# Autodesk Inventor assembly: A1
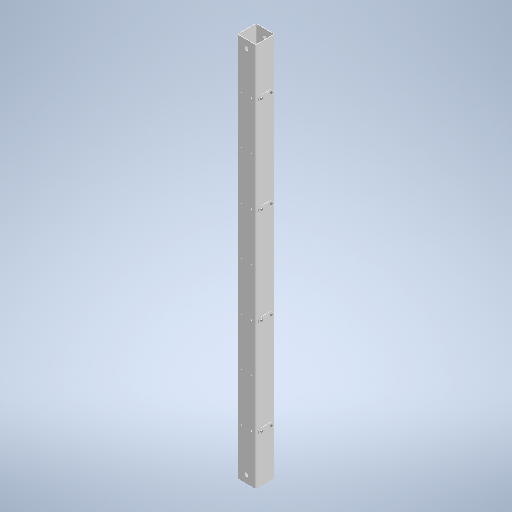
[picture p0: Inventor's stored thumbnail of the model, 512x512]
Saved by Autodesk Inventor 2025.2 (Build 292293000, 293)
## iProperties
Created: 2025-03-24
Part Number: A1
Document SubType Name: Assembly
Designer: Caspe
Author: Caspe
## Documents named in this file (6)
- C:\Users\Caspe\Documents\Semester 8\Project\Anomaly_Detection\Mechanical_Project\Inventor_project\A1.iam
- C:\Users\Caspe\Documents\Semester 8\Project\Anomaly_Detection\Mechanical_Project\Inventor_project\A1_Beam.ipt
- C:\Users\Caspe\Documents\Semester 8\Project\Anomaly_Detection\Mechanical_Project\Inventor_project\A1_joiners.ipt
- C:\Users\Caspe\Documents\Inventor\Content Center Files\R2025\en-US\Blind Rivet GB_T 12615.1-2004\Blind Rivet GB_T 12615.1-2004 3.2 X 10.5.ipt
- C:\Users\Caspe\Documents\Semester 8\Project\Anomaly_Detection\Mechanical_Project\Inventor_project\A1_joiners_MIR.ipt
- C:\Users\Caspe\Documents\Semester 8\Project\Anomaly_Detection\Mechanical_Project\Inventor_project\Leg_press_parameters.xlsx
## Components (26 placed, 4 different names)
1. A1_Beam:1 — Mate:1, Mate:2, Mate:3, Mate:4, Mate:6
2. A1_Beam:2 — Mate:1, Mate:2, Mate:3, Mate:5
3. A1_joiners_MIR:1 — Insert:2
4. A1_joiners_MIR:2
5. Blind Rivet GB/T 12615.1-2004 3.2 X 10.5:10
6. Blind Rivet GB/T 12615.1-2004 3.2 X 10.5:11
7. A1_joiners_MIR:3
8. Blind Rivet GB/T 12615.1-2004 3.2 X 10.5:12
9. Blind Rivet GB/T 12615.1-2004 3.2 X 10.5:13
10. A1_joiners_MIR:4
11. Blind Rivet GB/T 12615.1-2004 3.2 X 10.5:14
12. Blind Rivet GB/T 12615.1-2004 3.2 X 10.5:15
13. A1_joiners:1 — Mate:4, Mate:5, Mate:6, Insert:1
14. A1_joiners:2
15. A1_joiners:3
16. A1_joiners:4
17. Blind Rivet GB/T 12615.1-2004 3.2 X 10.5:9 — Insert:2
18. Blind Rivet GB/T 12615.1-2004 3.2 X 10.5:16
19. Blind Rivet GB/T 12615.1-2004 3.2 X 10.5:1 — Insert:1
20. Blind Rivet GB/T 12615.1-2004 3.2 X 10.5:2
21. Blind Rivet GB/T 12615.1-2004 3.2 X 10.5:3
22. Blind Rivet GB/T 12615.1-2004 3.2 X 10.5:4
23. Blind Rivet GB/T 12615.1-2004 3.2 X 10.5:5
24. Blind Rivet GB/T 12615.1-2004 3.2 X 10.5:6
25. Blind Rivet GB/T 12615.1-2004 3.2 X 10.5:7
26. Blind Rivet GB/T 12615.1-2004 3.2 X 10.5:8
## Component patterns: (4 elements, first: A1_joiners:1), (2 elements, first: Blind Rivet GB/T 12615.1-2004 3.2 X 10.5:9), (2 elements, first: Blind Rivet GB/T 12615.1-2004 3.2 X 10.5:1), Component Pattern 1:2 (2 elements), Component Pattern 1:3 (2 elements), Component Pattern 1:4 (2 elements)
## Relationships (9: Mate 6, Insert 2, Flush 1)
- Mate:1: A1_Beam:1 ↔ A1_Beam:2
- Mate:2: A1_Beam:1 ↔ A1_Beam:2
- Mate:3: A1_Beam:1 ↔ A1_Beam:2
- Mate:4: A1_Beam:1 ↔ A1_joiners:1
- Mate:5: A1_Beam:2 ↔ A1_joiners:1
- Mate:6: A1_Beam:1 ↔ A1_joiners:1
- Insert:1: A1_joiners:1 ↔ Blind Rivet GB/T 12615.1-2004 3.2 X 10.5:1
- Flush:1 (25 mm)
- Insert:2: A1_joiners_MIR:1 ↔ Blind Rivet GB/T 12615.1-2004 3.2 X 10.5:9
## Named parameters: A_length = 1000 mm, A_width = 50 mm, A_bend = 20 mm, A_connection_width = 40 mm, A_displacement = 500 mm, A_hole_height = 10 mm, A_hole_length = 40 mm, A_joint_diameter = 10 mm, A_height = 50 mm, A_joint_tolerance = 3 mm, l___________ = 0 mm, B_length = 700 mm, B_width = 50 mm, B_bend = 20 mm, B_connection_width = 40 mm, B_hole_height = 10 mm, B_hole_length = 40 mm, l__________ = 0 mm, C_length = 400 mm, C_width = 20 mm, C_height = 330 mm, l_________ = 0 mm, rivet_diameter = 3.35 mm, rivet_displacement = 250 mm, plate_thickness = 2 mm, l________ = 0 mm, B_hinge_holes_spacing = 50 mm, B_height = 50 mm, A_B_spacing = 2 mm, L_Piston_Bottom = 21 mm, L_Piston_Top = 25 mm
